# Autodesk Inventor assembly: metal lead
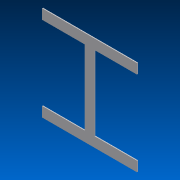
[picture p0: Inventor's stored thumbnail of the model, 180x180]
Saved by Autodesk Inventor 2012 (Build 160160000, 160)
## iProperties
Created: 2012-07-05
Part Number: metal lead
Document SubType Name: Assembly
Designer: Hemant
Author: Hemant
## Documents named in this file (3)
- C:\Users\Hemant\Documents\Battery Boxes\BB REAR A\Metal Lead\metal lead.iam
- C:\Users\Hemant\Documents\Battery Boxes\BB REAR A\Metal Lead\m1.ipt
- C:\Users\Hemant\Documents\Battery Boxes\BB REAR A\Metal Lead\m2.ipt
## Components (3 placed, 2 different names)
1. m2:1 — Mate:1, Flush:1, Mate:2
2. m1:1 — Mate:1, Mate:2
3. m1:2 — Flush:1
## Component patterns: (2 elements, first: m1:1)
## Relationships (3: Mate 2, Flush 1)
- Mate:1: m2:1 ↔ m1:1
- Flush:1: m2:1 ↔ m1:2
- Mate:2 (215.9 mm): m2:1 ↔ m1:1
